# Autodesk Inventor assembly: TS_V1_Fallmagazin_Schieber
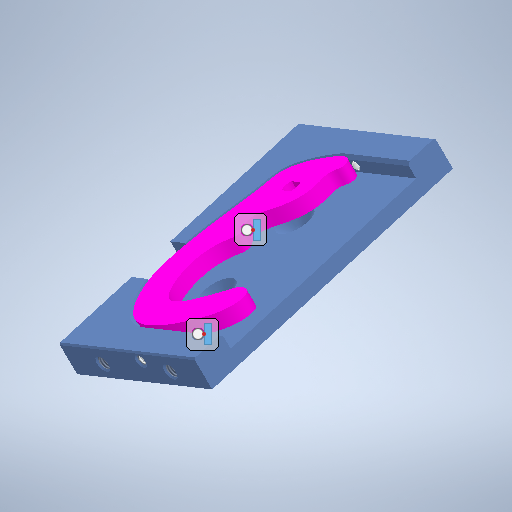
[picture p0: Inventor's stored thumbnail of the model, 512x512]
Saved by Autodesk Inventor 2025.2 (Build 292293000, 293)
## iProperties
Created: 2025-06-11
Part Number: TS_V1_Fallmagazin_Schieber
Document SubType Name: Assembly
Designer: tino
Author: tino
## Documents named in this file (4)
- C:\Users\tino\Documents_VM\Konstruieren_CAD\Useless Box\Eigene Bauteile\Fallmagazin\TS_V1_Fallmagazin_Schieber.iam
- C:\Users\tino\Documents_VM\Konstruieren_CAD\Useless Box\Eigene Bauteile\Fallmagazin\TS_V1_Fallmagazin_Schieber_int.ipt
- C:\Users\tino\Documents_VM\Konstruieren_CAD\Useless Box\_Useless_Box\Finger.ipt
- C:\Users\tino\Documents_VM\Konstruieren_CAD\Useless Box\Kaufteile\WUERTH_federndes_Druckstueck\Wuerth_5099201004_Federndes_Druckstueck,_Kugel,_Edelstahl_LOD_High\Wuerth_5099201004_Federndes_Druckstueck,_Kugel,_.iam
## Components (4 placed, 3 different names)
1. TS_V1_Fallmagazin_Schieber_int:1 — Passend:3, Passend:4, Passend:5
2. Finger:1 — Passend:3, Tangential:3, Tangential:4
3. Wuerth_5099201004_Federndes_Druckstueck,_Kugel,_:1 [sub-assembly] — Passend:4, Tangential:3
4. Wuerth_5099201004_Federndes_Druckstueck,_Kugel,_:2 [sub-assembly] — Passend:5, Tangential:4
## Relationships (7: Tangent 3, Mate 3, Angle 1)
- [Angle] (0 deg): TS_V1_Fallmagazin_Schieber_int:1 ↔ Finger:1
- [Tangent]: TS_V1_Fallmagazin_Schieber_int:1 ↔ Finger:1
- Passend:3 [Mate]: TS_V1_Fallmagazin_Schieber_int:1 ↔ Finger:1
- Passend:4 [Mate]: TS_V1_Fallmagazin_Schieber_int:1 ↔ Wuerth_5099201004_Federndes_Druckstueck,_Kugel,_:1
- Tangential:3: Finger:1 ↔ Wuerth_5099201004_Federndes_Druckstueck,_Kugel,_:1
- Passend:5 [Mate]: TS_V1_Fallmagazin_Schieber_int:1 ↔ Wuerth_5099201004_Federndes_Druckstueck,_Kugel,_:2
- Tangential:4: Finger:1 ↔ Wuerth_5099201004_Federndes_Druckstueck,_Kugel,_:2
